# Autodesk Inventor assembly: table
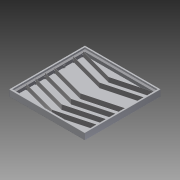
[picture p0: Inventor's stored thumbnail of the model, 180x180]
Saved by Autodesk Inventor 2013 (Build 170138000, 138)
## iProperties
Created: 2012-10-20
Part Number: table
Document SubType Name: Weldment
Designer: Istvan
Weld Material: Welded Aluminum-6061
Mass: 18318.1 g
Surface Area: 68009.8 cm^2
Volume: 8886.11 cm^3
Density: 2.06143 g/cm^3
Author: Istvan
## Documents named in this file (8)
- E:\GitHub\Crown-Fire\CAD\Frame\Table\table.iam
- E:\GitHub\Crown-Fire\CAD\Frame\Table\tableBottom.ipt
- E:\GitHub\Crown-Fire\CAD\Frame\Table\tableSide.ipt
- E:\GitHub\Crown-Fire\CAD\Frame\Table\slats.ipt
- E:\GitHub\Crown-Fire\CAD\Frame\Table\tableFrameLong.ipt
- E:\GitHub\Crown-Fire\CAD\Templates\squareTube1.5x2.ipt
- E:\GitHub\Crown-Fire\CAD\Frame\Table\slatHolder_r.iam
- E:\GitHub\Crown-Fire\CAD\Frame\Table\slatHolder_l.iam
## Components (15 placed, 6 different names)
1. tableBottom:1 — Mate:38, Mate:39, Mate:40, Mate:41, Mate:48, Mate:49, Mate:54, Mate:55, Mate:56, Mate:59, Mate:62, Mate:63, Mate:64, Mate:65, Mate:66, Mate:67
2. tableSide:1 — Mate:40, Mate:44, Mate:45, Mate:46, Mate:47, Mate:49, Mate:51
3. tableSide:2 — Mate:41, Mate:46, Mate:47, Mate:52, Mate:53, Mate:60
4. tableSide:3 — Mate:39, Mate:42, Mate:43, Mate:44, Mate:45, Mate:48, Mate:57
5. tableSide:4 — Mate:38, Mate:42, Mate:43, Mate:50
6. slats:1 — Tangent:4, Tangent:12, Mate:67, Mate:70
7. slats:2 — Tangent:5, Tangent:11, Mate:66, Mate:71
8. slats:3 — Tangent:7, Tangent:10, Mate:64, Mate:73
9. slats:4 — Tangent:6, Tangent:9, Mate:65, Mate:72
10. slats:6 — Tangent:3, Tangent:8, Mate:62, Mate:69
11. slats:7 — Tangent:1, Tangent:2, Mate:63, Mate:68
12. tableFrameLong:1 — Mate:51, Mate:52, Mate:55, Mate:58, Mate:61
13. tableFrameLong:2 — Mate:50, Mate:53, Mate:54
14. slatHolder_r:1 [sub-assembly] — Mate:56, Mate:57, Mate:58, Tangent:2, Tangent:8, Tangent:9, Tangent:10, Tangent:11, Tangent:12
15. slatHolder_l:1 [sub-assembly] — Mate:59, Mate:60, Mate:61, Tangent:1, Tangent:3, Tangent:4, Tangent:5, Tangent:6, Tangent:7, Mate:68, Mate:69, Mate:70, Mate:71, Mate:72, Mate:73
## Relationships (48: Mate 36, Tangent 12)
- Mate:38: tableBottom:1 ↔ tableSide:4
- Mate:39: tableBottom:1 ↔ tableSide:3
- Mate:40: tableBottom:1 ↔ tableSide:1
- Mate:41: tableBottom:1 ↔ tableSide:2
- Mate:42: tableSide:3 ↔ tableSide:4
- Mate:43: tableSide:3 ↔ tableSide:4
- Mate:44: tableSide:1 ↔ tableSide:3
- Mate:45: tableSide:1 ↔ tableSide:3
- Mate:46: tableSide:1 ↔ tableSide:2
- Mate:47: tableSide:1 ↔ tableSide:2
- Mate:48: tableBottom:1 ↔ tableSide:3
- Mate:49: tableBottom:1 ↔ tableSide:1
- Mate:50: tableSide:4 ↔ tableFrameLong:2
- Mate:51: tableSide:1 ↔ tableFrameLong:1
- Mate:52: tableSide:2 ↔ tableFrameLong:1
- Mate:53: tableSide:2 ↔ tableFrameLong:2
- Mate:54: tableBottom:1 ↔ tableFrameLong:2
- Mate:55: tableBottom:1 ↔ tableFrameLong:1
- Mate:56: tableBottom:1 ↔ slatHolder_r:1
- Mate:57: tableSide:3 ↔ slatHolder_r:1
- Mate:58: tableFrameLong:1 ↔ slatHolder_r:1
- Mate:59: tableBottom:1 ↔ slatHolder_l:1
- Mate:60: tableSide:2 ↔ slatHolder_l:1
- Mate:61: tableFrameLong:1 ↔ slatHolder_l:1
- Tangent:1: slats:7 ↔ slatHolder_l:1
- Tangent:2: slats:7 ↔ slatHolder_r:1
- Tangent:3: slats:6 ↔ slatHolder_l:1
- Tangent:4: slats:1 ↔ slatHolder_l:1
- Tangent:5: slats:2 ↔ slatHolder_l:1
- Tangent:6: slats:4 ↔ slatHolder_l:1
- Tangent:7: slats:3 ↔ slatHolder_l:1
- Tangent:8: slats:6 ↔ slatHolder_r:1
- Mate:62: tableBottom:1 ↔ slats:6
- Mate:63: tableBottom:1 ↔ slats:7
- Tangent:9: slats:4 ↔ slatHolder_r:1
- Mate:65: tableBottom:1 ↔ slats:4
- Tangent:10: slats:3 ↔ slatHolder_r:1
- Mate:64: tableBottom:1 ↔ slats:3
- Tangent:11: slats:2 ↔ slatHolder_r:1
- Mate:66: tableBottom:1 ↔ slats:2
- Tangent:12: slats:1 ↔ slatHolder_r:1
- Mate:67: tableBottom:1 ↔ slats:1
- Mate:68: slats:7 ↔ slatHolder_l:1
- Mate:69: slats:6 ↔ slatHolder_l:1
- Mate:70: slats:1 ↔ slatHolder_l:1
- Mate:71: slats:2 ↔ slatHolder_l:1
- Mate:72: slats:4 ↔ slatHolder_l:1
- Mate:73: slats:3 ↔ slatHolder_l:1
